# Autodesk Inventor assembly: Mecanum_Wheel_60mm_Right_ASM_AP214
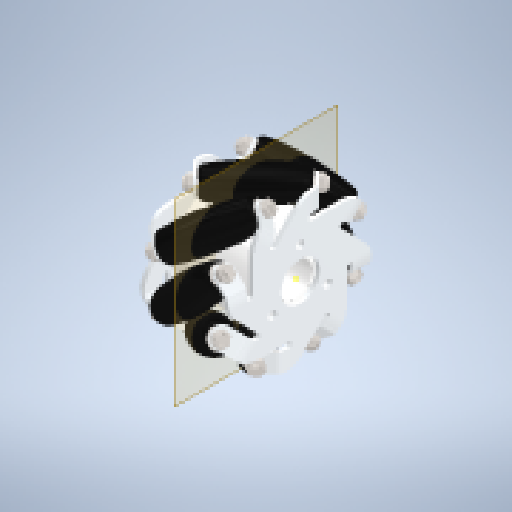
[picture p0: Inventor's stored thumbnail of the model, 512x512]
Saved by Autodesk Inventor 2023 (Build 270158000, 158)
## iProperties
Created: 2015-10-21
Part Number: Mecanum_Wheel_60mm_Right_ASM_AP214
Description: STEP AP214
Document SubType Name: Assembly
Designer: Khasal
Title: Mecanum_Wheel_60mm_Right_ASM_AP214.STEP
Revision Number: ANY
## Documents named in this file (7)
- C:\GoogleDrive\Cloud\Мой диск\Projects\Botik v0.1\wheel assembly\Mecanum Wheel (dia 60) Left\Mecanum_Wheel_60mm_Right_ASM_AP214.iam
- C:\GoogleDrive\Cloud\Мой диск\Projects\Botik v0.1\wheel assembly\Mecanum Wheel (dia 60) Left\plate_2_Varsayilan.ipt
- C:\GoogleDrive\Cloud\Мой диск\Projects\Botik v0.1\wheel assembly\Mecanum Wheel (dia 60) Left\roller_Varsayilan.ipt
- C:\GoogleDrive\Cloud\Мой диск\Projects\Botik v0.1\wheel assembly\Mecanum Wheel (dia 60) Left\liner_Varsayilan.ipt
- C:\GoogleDrive\Cloud\Мой диск\Projects\Botik v0.1\wheel assembly\Mecanum Wheel (dia 60) Left\inner_cylinder_Varsayilan.ipt
- C:\GoogleDrive\Cloud\Мой диск\Projects\Botik v0.1\wheel assembly\Mecanum Wheel (dia 60) Left\two_sided_screw_Varsayilan.ipt
- C:\GoogleDrive\Cloud\Мой диск\Projects\Botik v0.1\wheel assembly\Mecanum Wheel (dia 60) Left\3mm_bolt_Varsayilan.ipt
## Components (51 placed, 51 different names)
1. plate_2_Varsayilan_1 — Симметрия:1
2. plate_2_Varsayilan_2 — Симметрия:1
3. roller_Varsayilan_3
4. liner_Varsayilan_4
5. liner_Varsayilan_5
6. inner_cylinder_Varsayilan_6
7. two_sided_screw_Varsayilan_7
8. 3mm_bolt_Varsayilan_8
9. 3mm_bolt_Varsayilan_9
10. two_sided_screw_Varsayilan_16
11. two_sided_screw_Varsayilan_17
12. two_sided_screw_Varsayilan_18
13. two_sided_screw_Varsayilan_19
14. two_sided_screw_Varsayilan_20
15. two_sided_screw_Varsayilan_21
16. two_sided_screw_Varsayilan_22
17. 3mm_bolt_Varsayilan_23
18. 3mm_bolt_Varsayilan_24
19. 3mm_bolt_Varsayilan_25
20. 3mm_bolt_Varsayilan_26
21. 3mm_bolt_Varsayilan_27
22. 3mm_bolt_Varsayilan_28
23. 3mm_bolt_Varsayilan_29
24. 3mm_bolt_Varsayilan_30
25. 3mm_bolt_Varsayilan_31
26. 3mm_bolt_Varsayilan_32
27. 3mm_bolt_Varsayilan_33
28. 3mm_bolt_Varsayilan_34
29. 3mm_bolt_Varsayilan_35
30. 3mm_bolt_Varsayilan_36
31. liner_Varsayilan_37
32. liner_Varsayilan_38
33. liner_Varsayilan_39
34. liner_Varsayilan_40
35. liner_Varsayilan_41
36. liner_Varsayilan_42
37. liner_Varsayilan_43
38. liner_Varsayilan_44
39. liner_Varsayilan_45
40. liner_Varsayilan_46
41. liner_Varsayilan_47
42. liner_Varsayilan_48
43. liner_Varsayilan_49
44. liner_Varsayilan_50
45. roller_Varsayilan_51
46. roller_Varsayilan_52
47. roller_Varsayilan_53
48. roller_Varsayilan_54
49. roller_Varsayilan_55
50. roller_Varsayilan_56
51. roller_Varsayilan_57
## Relationships (1: Symmetry 1)
- Симметрия:1 [Symmetry]: plate_2_Varsayilan_1 ↔ plate_2_Varsayilan_2
